# Autodesk Inventor assembly: TheLightWithinYou-Assembly-V3
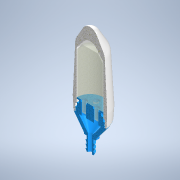
[picture p0: Inventor's stored thumbnail of the model, 180x180]
Saved by Autodesk Inventor 2021 (Build 250183000, 183)
## iProperties
Created: 2021-08-12
Part Number: TheLightWithinYou-Assembly-V3
Document SubType Name: Assembly
Designer: incep
Author: incep
## Documents named in this file (4)
- C:\Users\incep\Desktop\3D Printer Stuff\TheLightWithinYou\TheLightWithinYou-Assembly-V3.iam
- C:\Users\incep\Desktop\3D Printer Stuff\TheLightWithinYou\Upper-Threaded-v2.ipt
- C:\Users\incep\Desktop\3D Printer Stuff\TheLightWithinYou\Bottom-V3.ipt
- C:\Users\incep\Desktop\3D Printer Stuff\TheLightWithinYou\Flashbulb.ipt
## Components (3 placed, 3 different names)
1. Upper-Threaded-v2:1 — Mate:1, Mate:2, Mate:3
2. Bottom-V3:1 — Mate:1, Mate:2, Mate:4, Mate:5, Mate:6
3. Flashbulb:1 — Mate:4, Mate:5, Mate:6
## Relationships (6: Mate 6)
- Mate:1: Upper-Threaded-v2:1 ↔ Bottom-V3:1
- Mate:2: Upper-Threaded-v2:1 ↔ Bottom-V3:1
- Mate:3: Upper-Threaded-v2:1
- Mate:4: Bottom-V3:1 ↔ Flashbulb:1
- Mate:5: Bottom-V3:1 ↔ Flashbulb:1
- Mate:6: Bottom-V3:1 ↔ Flashbulb:1
